# Autodesk Inventor assembly: CE-7.1.1_CE-2.1.4_LY
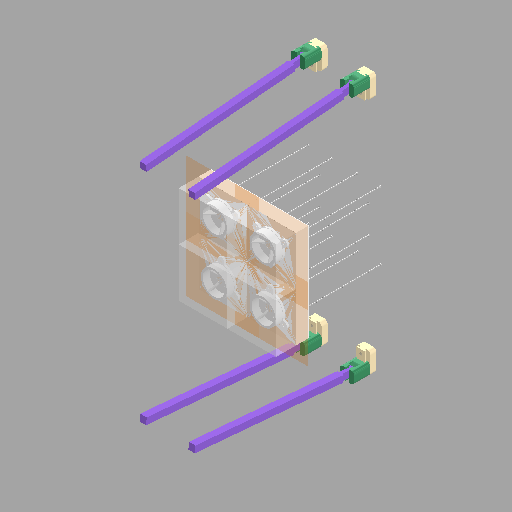
[picture p0: Inventor's stored thumbnail of the model, 512x512]
Saved by Autodesk Inventor 2024 (Build 280153000, 153)
## iProperties
Created: 2024-02-25
Part Number: CE-7.1.1_CE-2.1.4_LY
Document SubType Name: Assembly
Designer: Alex
Author: Alex
## Documents named in this file (2)
- C:\Shared\alex-bartella-schoolwork\4z03\Week 6\CE-7.1.1_CE-2.1.4_LY.iam
- C:\Shared\alex-bartella-schoolwork\4z03\Week 6\CE-7.1.1_CE-2.1.4_PZ.iam
## Components (4 placed, 1 different names)
1. CE-7.1.1_CE-2.1.4_PZ:1 [sub-assembly] — Flush:1, Flush:2, Flush:3
2. CE-7.1.1_CE-2.1.4_PZ:2 [sub-assembly] — Flush:4, Flush:5, Flush:6
3. CE-7.1.1_CE-2.1.4_PZ:3 [sub-assembly] — Flush:7, Flush:8, Flush:9
4. CE-7.1.1_CE-2.1.4_PZ:4 [sub-assembly] — Flush:10, Flush:11, Flush:12
## Relationships (13: Flush 13)
- Flush:1: CE-7.1.1_CE-2.1.4_PZ:1
- Flush:2: CE-7.1.1_CE-2.1.4_PZ:1
- Flush:3: CE-7.1.1_CE-2.1.4_PZ:1
- Flush:4: CE-7.1.1_CE-2.1.4_PZ:2
- Flush:5: CE-7.1.1_CE-2.1.4_PZ:2
- Flush:6: CE-7.1.1_CE-2.1.4_PZ:2
- Flush:7: CE-7.1.1_CE-2.1.4_PZ:3
- Flush:8: CE-7.1.1_CE-2.1.4_PZ:3
- Flush:9: CE-7.1.1_CE-2.1.4_PZ:3
- Flush:10: CE-7.1.1_CE-2.1.4_PZ:4
- Flush:11: CE-7.1.1_CE-2.1.4_PZ:4
- Flush:12: CE-7.1.1_CE-2.1.4_PZ:4
- Flush:13 (-5.5 mm)
